# Autodesk Inventor assembly: Raspberry Pi 3
(part 2 of 2)
357. Raspberry Pi 3163:3
358. Raspberry Pi 3164:3
359. Solder2:1
360. Solder2:41
361. Solder2:42
362. Solder2:43
363. Solder2:44
364. Solder2:45
365. Solder2:46
366. Solder2:47
367. Solder2:48
368. Solder2:49
369. Solder2:59
370. Raspberry Pi 3358:1
371. Raspberry Pi 3359:1
372. Solder2:68
373. Solder2:69
374. Solder2:70
375. Solder2:71
376. Solder2:72
377. Solder2:73
378. Solder2:74
379. Solder2:75
380. Solder2:76
381. Solder2:77
382. Solder2:78
383. Solder2:79
384. mf-msmf050-2:1
385. Solder2:87
386. Raspberry Pi 3163:4
387. Raspberry Pi 353:4
388. Raspberry Pi 3164:4
389. Raspberry Pi 3165:4
390. Raspberry Pi 3163:5
391. Raspberry Pi 353:5
392. Raspberry Pi 3164:5
393. Raspberry Pi 3165:5
394. Raspberry Pi 3163:6
395. Raspberry Pi 353:6
396. Raspberry Pi 3164:6
397. Raspberry Pi 3165:6
398. Raspberry Pi 3141:3
399. Raspberry Pi 3141:4
400. Raspberry Pi 3141:5
401. Raspberry Pi 3141:6
402. Raspberry Pi 3141:7
403. Raspberry Pi 3141:8
404. Raspberry Pi 3141:9
405. Raspberry Pi 3141:10
406. Raspberry Pi 3141:11
407. Raspberry Pi 3141:12
408. Raspberry Pi 3141:13
409. Raspberry Pi 3141:14
410. Raspberry Pi 3141:15
411. Raspberry Pi 3141:17
412. Raspberry Pi 3141:18
413. Raspberry Pi 3141:19
414. Raspberry Pi 3141:20
415. Raspberry Pi 3141:21
416. Raspberry Pi 3141:22
417. Raspberry Pi 3141:23
418. Raspberry Pi 3141:24
419. Raspberry Pi 3141:25
420. Raspberry Pi 3141:26
421. Raspberry Pi 3141:27
422. Raspberry Pi 3141:28
423. Raspberry Pi 3141:29
424. Raspberry Pi 3141:30
425. Raspberry Pi 3141:31
426. Raspberry Pi 3141:32
427. Raspberry Pi 3141:35
428. Raspberry Pi 3141:36
429. Raspberry Pi 3141:37
430. Raspberry Pi 3141:38
431. Raspberry Pi 3141:39
432. Raspberry Pi 3141:40
433. Raspberry Pi 3141:41
434. Raspberry Pi 3141:42
435. Raspberry Pi 3141:43
436. Raspberry Pi 3141:44
437. Raspberry Pi 3141:45
438. Raspberry Pi 3141:46
439. Raspberry Pi 3141:47
440. Raspberry Pi 3141:48
441. Raspberry Pi 3141:49
442. Raspberry Pi 3141:50
443. Raspberry Pi 3141:51
444. Raspberry Pi 3141:52
445. Raspberry Pi 3141:53
446. Raspberry Pi 3141:54
447. Raspberry Pi 3141:55
448. Raspberry Pi 3141:56
449. Raspberry Pi 3141:57
450. Raspberry Pi 3141:58
451. Raspberry Pi 3141:59
452. Raspberry Pi 3141:60
453. Raspberry Pi 3141:61
454. Raspberry Pi 3141:62
455. Raspberry Pi 3141:63
456. Raspberry Pi 374:6
457. Raspberry Pi 3141:66
458. Raspberry Pi 3141:67
459. Raspberry Pi 3141:68
460. Raspberry Pi 3141:69
461. Raspberry Pi 3141:70
462. Raspberry Pi 3141:72
463. Raspberry Pi 3141:73
464. Raspberry Pi 3141:74
465. Raspberry Pi 3141:75
466. Raspberry Pi 3141:76
467. Raspberry Pi 3141:77
468. Raspberry Pi 3141:78
469. Raspberry Pi 3141:79
470. Raspberry Pi 3141:80
471. Raspberry Pi 3141:82
472. Raspberry Pi 3141:84
473. Raspberry Pi 3141:86
474. Raspberry Pi 3141:88
475. Raspberry Pi 3141:89
476. Raspberry Pi 3141:90
477. Raspberry Pi 3141:91
478. Raspberry Pi 3141:92
479. Raspberry Pi 3141:93
480. Raspberry Pi 3141:95
481. Raspberry Pi 3141:96
482. Raspberry Pi 3141:97
483. Raspberry Pi 3141:98
484. Raspberry Pi 3141:100
485. Raspberry Pi 3141:101
486. Raspberry Pi 3141:102
487. Raspberry Pi 3141:103
488. Raspberry Pi 3141:104
489. Raspberry Pi 3141:105
490. Raspberry Pi 3141:106
491. Raspberry Pi 3141:107
492. Raspberry Pi 3141:108
493. Raspberry Pi 3141:109
494. Raspberry Pi 3141:110
495. Raspberry Pi 3141:112
496. Raspberry Pi 3141:113
497. Raspberry Pi 3141:114
498. Raspberry Pi 3141:115
499. Raspberry Pi 3141:116
500. Raspberry Pi 3141:117
501. Raspberry Pi 3141:118
502. Raspberry Pi 3141:119
503. Raspberry Pi 3141:120
504. Raspberry Pi 3141:121
505. Raspberry Pi 3141:122
506. Raspberry Pi 3141:123
507. Raspberry Pi 3141:124
508. Raspberry Pi 3141:126
509. Raspberry Pi 3281:2
510. Raspberry Pi 3280:2
511. Raspberry Pi 3282:2
512. Raspberry Pi 3285:2
513. Raspberry Pi 3283:2
514. Raspberry Pi 3284:2
515. Raspberry Pi 34:2
516. Raspberry Pi 3141:128
517. Raspberry Pi 3141:129
518. Raspberry Pi 3141:130
519. Raspberry Pi 3141:131
520. Raspberry Pi 3141:132
521. Raspberry Pi 3141:133
522. Raspberry Pi 3141:134
523. Raspberry Pi 3141:135
524. Raspberry Pi 3141:137
525. Raspberry Pi 3141:138
526. Raspberry Pi 3141:139
527. Raspberry Pi 3141:140
528. Raspberry Pi 3141:141
529. Raspberry Pi 3141:143
530. Raspberry Pi 3141:145
531. Raspberry Pi 345:2
532. Raspberry Pi 345:3
533. Raspberry Pi 345:4
534. Raspberry Pi 345:5
535. Assem1^Raspberry Pi 3:1 [sub-assembly]
536. Raspberry Pi 3141:147
537. Solder2:2
538. Solder2:3
539. Solder2:4
540. Solder2:5
541. Solder2:6
542. Solder2:7
543. Solder2:8
544. Solder2:9
545. Solder2:10
546. Solder2:11
547. Solder2:12
548. Solder2:13
549. Solder2:14
550. Solder2:15
551. Solder2:16
552. Solder2:17
553. Solder2:18
554. Solder2:19
555. Solder2:20
556. Solder2:21
557. Solder2:22
558. Solder2:23
559. Solder2:24
560. Solder2:25
561. Solder2:26
562. Solder2:27
563. Solder2:28
564. Solder2:29
565. Solder2:30
566. Solder2:31
567. Solder2:32
568. Solder2:33
569. Solder2:34
570. Solder2:35
571. Solder2:36
572. Solder2:37
573. Solder2:38
574. Solder2:39
575. Solder2:40
576. Solder2:51
577. Solder2:52
578. Solder2:53
579. Solder2:54
580. Solder2:55
581. Solder2:56
582. Solder2:57
583. Solder2:61
584. Solder2:62
585. Solder2:63
586. Solder2:64
587. Solder2:65
588. Solder2:66
589. Solder2:67
590. Solder2:81
591. Solder2:82
592. Solder2:83
593. Solder2:84
594. Solder2:85
595. Solder2:86
596. raspberry_pi_B+_(microsd2):1
597. Raspberry Pi 3242:2
598. Raspberry Pi 3242:3
599. Raspberry Pi 3242:4
600. Raspberry Pi 3242:5
601. Raspberry Pi 3242:6
602. Raspberry Pi 3242:7
603. Raspberry Pi 3242:8
604. Raspberry Pi 3242:9
605. Raspberry Pi 3242:10
606. Raspberry Pi 3242:11
607. Raspberry Pi 3242:12
608. Raspberry Pi 3242:13
609. Raspberry Pi 3242:14
610. Raspberry Pi 3242:15
611. Raspberry Pi 3242:16
612. Raspberry Pi 3242:17
613. Raspberry Pi 3242:18
614. Raspberry Pi 3242:19
615. Raspberry Pi 3242:20
616. Raspberry Pi 3266:2
617. Raspberry Pi 3266:3
618. Raspberry Pi 3266:4
619. Raspberry Pi 3266:5
620. Raspberry Pi 3266:6
621. Raspberry Pi 3266:7
622. Raspberry Pi 3266:8
623. Raspberry Pi 3266:9
624. Raspberry Pi 3266:10
625. Raspberry Pi 3266:11
626. Raspberry Pi 3266:12
627. Raspberry Pi 3266:13
628. Raspberry Pi 3266:14
629. Raspberry Pi 3266:15
630. Raspberry Pi 3266:16
631. Raspberry Pi 3266:17
632. Raspberry Pi 3266:18
633. Raspberry Pi 3266:19
634. Raspberry Pi 3266:20
